# Autodesk Inventor assembly: Lift
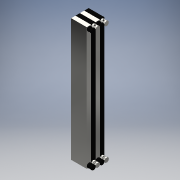
[picture p0: Inventor's stored thumbnail of the model, 180x180]
Saved by Autodesk Inventor 2016 (Build 200138000, 138)
## iProperties
Created: 2017-02-01
Part Number: Lift
Document SubType Name: Assembly
Designer: RoboticsUser
Author: RoboticsUser
## Documents named in this file (3)
- C:\Robotics\CAD\2016-17_CAD\Lift.iam
- C:\Robotics\CAD\2016-17_CAD\LiftSlidePart.ipt
- C:\Robotics\CAD\2016-17_CAD\LiftPully.ipt
## Components (12 placed, 2 different names)
1. LiftSlidePart:1 — Mate:1, Tangent:1, Tangent:2, Mate:5, Flush:1, Flush:2, Tangent:10, Mate:9, Tangent:11, Tangent:12
2. LiftSlidePart:2 — Mate:2, Tangent:3, Tangent:4, Mate:5, Flush:1, Flush:2, Mate:6, Flush:3, Flush:4, Mate:8, Tangent:9, Tangent:14
3. LiftSlidePart:3 — Mate:3, Tangent:5, Tangent:6, Mate:6, Flush:3, Flush:4, Mate:7, Flush:5, Flush:6, Mate:10, Tangent:13
4. LiftSlidePart:4 — Mate:4, Tangent:7, Tangent:8, Mate:7, Flush:5, Flush:6, Mate:11, Tangent:15, Tangent:16
5. LiftPully:1 — Mate:2, Tangent:3, Tangent:4
6. LiftPully:2 — Mate:3, Tangent:5, Tangent:6
7. LiftPully:3 — Mate:1, Tangent:1, Tangent:2
8. LiftPully:4 — Mate:4, Tangent:7, Tangent:8
9. LiftPully:5 — Mate:10, Tangent:13, Tangent:14
10. LiftPully:6 — Mate:11, Tangent:15, Tangent:16
11. LiftPully:7 — Mate:9, Tangent:11, Tangent:12
12. LiftPully:8 — Mate:8, Tangent:9, Tangent:10
## Relationships (33: Tangent 16, Mate 11, Flush 6)
- Mate:1: LiftSlidePart:1 ↔ LiftPully:3
- Tangent:1: LiftSlidePart:1 ↔ LiftPully:3
- Mate:2: LiftSlidePart:2 ↔ LiftPully:1
- Tangent:2: LiftSlidePart:1 ↔ LiftPully:3
- Tangent:3: LiftSlidePart:2 ↔ LiftPully:1
- Tangent:4: LiftSlidePart:2 ↔ LiftPully:1
- Mate:3: LiftSlidePart:3 ↔ LiftPully:2
- Tangent:5: LiftSlidePart:3 ↔ LiftPully:2
- Tangent:6: LiftSlidePart:3 ↔ LiftPully:2
- Mate:4: LiftSlidePart:4 ↔ LiftPully:4
- Tangent:7: LiftSlidePart:4 ↔ LiftPully:4
- Tangent:8: LiftSlidePart:4 ↔ LiftPully:4
- Mate:5: LiftSlidePart:1 ↔ LiftSlidePart:2
- Flush:1: LiftSlidePart:1 ↔ LiftSlidePart:2
- Flush:2: LiftSlidePart:1 ↔ LiftSlidePart:2
- Mate:6: LiftSlidePart:2 ↔ LiftSlidePart:3
- Flush:3: LiftSlidePart:2 ↔ LiftSlidePart:3
- Flush:4: LiftSlidePart:2 ↔ LiftSlidePart:3
- Mate:7: LiftSlidePart:3 ↔ LiftSlidePart:4
- Flush:5: LiftSlidePart:3 ↔ LiftSlidePart:4
- Flush:6: LiftSlidePart:3 ↔ LiftSlidePart:4
- Mate:8: LiftSlidePart:2 ↔ LiftPully:8
- Tangent:9: LiftSlidePart:2 ↔ LiftPully:8
- Tangent:10: LiftSlidePart:1 ↔ LiftPully:8
- Mate:9: LiftSlidePart:1 ↔ LiftPully:7
- Tangent:11: LiftSlidePart:1 ↔ LiftPully:7
- Tangent:12: LiftSlidePart:1 ↔ LiftPully:7
- Mate:10: LiftSlidePart:3 ↔ LiftPully:5
- Tangent:13: LiftSlidePart:3 ↔ LiftPully:5
- Tangent:14: LiftSlidePart:2 ↔ LiftPully:5
- Mate:11: LiftSlidePart:4 ↔ LiftPully:6
- Tangent:15: LiftSlidePart:4 ↔ LiftPully:6
- Tangent:16: LiftSlidePart:4 ↔ LiftPully:6
